# Autodesk Inventor assembly: Kinect
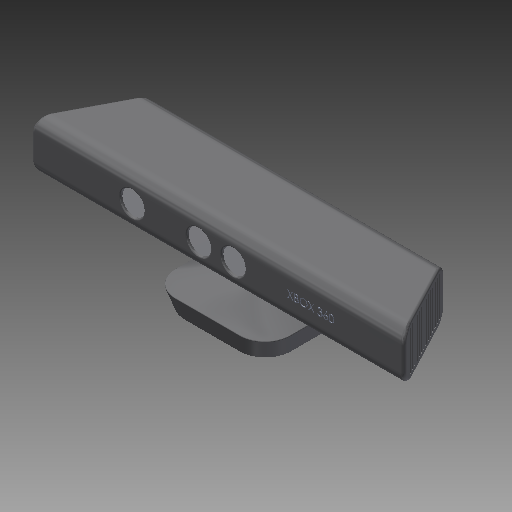
[picture p0: Inventor's stored thumbnail of the model, 512x512]
Saved by Autodesk Inventor 2018 (Build 220112000, 112)
## iProperties
Created: 2013-10-22
Part Number: Kinect
Description: STEP AP214
Document SubType Name: Assembly
Designer: snipe
Sending System: SolidWorks 2014
Preprocessor: SwSTEP 2.0
Title: Kinect.STEP
Revision Number: TUTTO
## Documents named in this file (3)
- F:\Clark\Assets\Kinect.iam
- C:\Users\snipe\Downloads\base KINECT.ipt
- C:\Users\snipe\Downloads\KINECT XBOX.ipt
## Components (2 placed, 2 different names)
1. base KINECT_1 — Flush:1, Mate:1, Mate:2
2. KINECT XBOX_2 — Flush:1, Mate:1, Angle:1, Angle:2
## Relationships (5: Mate 2, Angle 2, Flush 1)
- Flush:1: base KINECT_1 ↔ KINECT XBOX_2
- Mate:1: base KINECT_1 ↔ KINECT XBOX_2
- Mate:2: base KINECT_1
- Angle:1 (0 deg): KINECT XBOX_2
- Angle:2 (0 deg): KINECT XBOX_2
